# Autodesk Inventor assembly: (FINAL) 1QUAD WITH HARDWARE
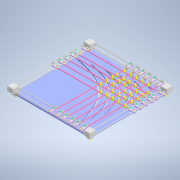
[picture p0: Inventor's stored thumbnail of the model, 180x180]
Saved by Autodesk Inventor 2022 (Build 260153000, 153)
## iProperties
Created: 2022-11-16
Part Number: (FINAL) 1QUAD WITH HARDWARE
Document SubType Name: Assembly
Designer: matia
Author: matia
## Documents named in this file (7)
- C:\Users\matia\Desktop\(V2) FULL ASSEMBLY\(FINAL) 1QUAD WITH HARDWARE.iam
- C:\Users\matia\Desktop\(V2) FULL ASSEMBLY\One quadrant Board.ipt
- C:\Users\matia\Desktop\(V2) FULL ASSEMBLY\bar.ipt
- C:\Users\matia\Desktop\(V2) FULL ASSEMBLY\(FINAL)2SIDEROLLER.iam
- C:\Users\matia\Desktop\(V2) FULL ASSEMBLY\newblockwithnopeg.ipt
- C:\Users\matia\Desktop\(V2) FULL ASSEMBLY\(FINAL) CORNER LH.iam
- C:\Users\matia\Desktop\(V2) FULL ASSEMBLY\(FINAL) CORNER RH.iam
## Components (55 placed, 6 different names)
1. One quadrant Board:1 — Mate:50, Mate:51, Mate:56, Mate:57, Mate:62, Mate:63, Mate:64, Mate:65
2. bar:1 — Mate:69, Mate:70
3. bar:2 — Mate:27, Mate:29, Mate:31, Mate:33, Mate:35, Mate:37, Mate:66, Mate:67
4. bar:3 — Mate:71, Mate:72
5. bar:4 — Mate:26, Mate:28, Mate:30, Mate:32, Mate:34, Mate:36, Mate:68, Mate:84, Mate:85
6. bar:5 — Mate:38, Mate:40, Mate:42, Mate:44, Mate:46, Mate:48, Mate:59, Mate:60
7. bar:6 — Mate:39, Mate:41, Mate:43, Mate:45, Mate:47, Mate:49, Mate:58, Mate:61
8. bar:7 — Mate:52, Mate:53
9. bar:8 — Mate:54, Mate:55
10. (FINAL)2SIDEROLLER:1 [sub-assembly] — Mate:26, Mate:27, Mate:80, Mate:100, Mate:110, Mate:114, Mate:134
11. (FINAL)2SIDEROLLER:2 [sub-assembly] — Mate:34, Mate:35, Mate:78, Mate:98, Mate:112, Mate:130, Mate:132
12. (FINAL)2SIDEROLLER:3 [sub-assembly] — Mate:36, Mate:37, Mate:82, Mate:102, Mate:104, Mate:106, Mate:108
13. (FINAL)2SIDEROLLER:4 [sub-assembly] — Mate:32, Mate:33, Mate:86, Mate:88, Mate:90, Mate:92, Mate:94
14. (FINAL)2SIDEROLLER:5 [sub-assembly] — Mate:30, Mate:31, Mate:74, Mate:116, Mate:118, Mate:120, Mate:122
15. (FINAL)2SIDEROLLER:6 [sub-assembly] — Mate:28, Mate:29, Mate:76, Mate:96, Mate:124, Mate:126, Mate:128
16. (FINAL)2SIDEROLLER:7 [sub-assembly] — Mate:38, Mate:39, Mate:87, Mate:103, Mate:109, Mate:111, Mate:115
17. (FINAL)2SIDEROLLER:8 [sub-assembly] — Mate:40, Mate:41, Mate:91, Mate:107, Mate:119, Mate:125, Mate:131
18. (FINAL)2SIDEROLLER:9 [sub-assembly] — Mate:42, Mate:43, Mate:93, Mate:121, Mate:127, Mate:129, Mate:133
19. (FINAL)2SIDEROLLER:10 [sub-assembly] — Mate:44, Mate:45, Mate:83, Mate:95, Mate:97, Mate:99, Mate:101
20. (FINAL)2SIDEROLLER:11 [sub-assembly] — Mate:46, Mate:47, Mate:89, Mate:105, Mate:113, Mate:117, Mate:123
21. (FINAL)2SIDEROLLER:12 [sub-assembly] — Mate:48, Mate:49, Mate:73, Mate:75, Mate:77, Mate:79, Mate:81
22. newblockwithnopeg:1 — Mate:73, Mate:74
23. (FINAL) CORNER LH:2 [sub-assembly] — Mate:56, Mate:57, Mate:58, Mate:59, Mate:60, Mate:61
24. (FINAL) CORNER LH:3 [sub-assembly] — Mate:64, Mate:65, Mate:69, Mate:70, Mate:71, Mate:72
25. (FINAL) CORNER RH:1 [sub-assembly] — Mate:50, Mate:51, Mate:52, Mate:53, Mate:54, Mate:55
26. (FINAL) CORNER RH:2 [sub-assembly] — Mate:62, Mate:63, Mate:66, Mate:67, Mate:68, Mate:84, Mate:85
27. newblockwithnopeg:2 — Mate:75, Mate:76
28. newblockwithnopeg:3 — Mate:81, Mate:82
29. newblockwithnopeg:4 — Mate:79, Mate:80
30. newblockwithnopeg:5 — Mate:77, Mate:78
31. newblockwithnopeg:6 — Mate:83, Mate:86
32. newblockwithnopeg:7 — Mate:87, Mate:88
33. newblockwithnopeg:8 — Mate:91, Mate:92
34. newblockwithnopeg:9 — Mate:89, Mate:90
35. newblockwithnopeg:10 — Mate:93, Mate:94
36. newblockwithnopeg:11 — Mate:95, Mate:96
37. newblockwithnopeg:12 — Mate:99, Mate:100
38. newblockwithnopeg:13 — Mate:97, Mate:98
39. newblockwithnopeg:14 — Mate:101, Mate:102
40. newblockwithnopeg:15 — Mate:103, Mate:104
41. newblockwithnopeg:16 — Mate:105, Mate:106
42. newblockwithnopeg:17 — Mate:115, Mate:116
43. newblockwithnopeg:18 — Mate:121, Mate:122
44. newblockwithnopeg:19 — Mate:125, Mate:126
45. newblockwithnopeg:20 — Mate:123, Mate:124
46. newblockwithnopeg:21 — Mate:119, Mate:120
47. newblockwithnopeg:22 — Mate:117, Mate:118
48. newblockwithnopeg:23 — Mate:113, Mate:114
49. newblockwithnopeg:24 — Mate:111, Mate:112
50. newblockwithnopeg:25 — Mate:109, Mate:110
51. newblockwithnopeg:26 — Mate:107, Mate:108
52. newblockwithnopeg:27 — Mate:133, Mate:134
53. newblockwithnopeg:28 — Mate:131, Mate:132
54. newblockwithnopeg:29 — Mate:129, Mate:130
55. newblockwithnopeg:30 — Mate:127, Mate:128
## Relationships (109: Mate 109)
- Mate:26: bar:4 ↔ (FINAL)2SIDEROLLER:1
- Mate:27: bar:2 ↔ (FINAL)2SIDEROLLER:1
- Mate:28: bar:4 ↔ (FINAL)2SIDEROLLER:6
- Mate:29: bar:2 ↔ (FINAL)2SIDEROLLER:6
- Mate:30: bar:4 ↔ (FINAL)2SIDEROLLER:5
- Mate:31: bar:2 ↔ (FINAL)2SIDEROLLER:5
- Mate:32: bar:4 ↔ (FINAL)2SIDEROLLER:4
- Mate:33: bar:2 ↔ (FINAL)2SIDEROLLER:4
- Mate:34: bar:4 ↔ (FINAL)2SIDEROLLER:2
- Mate:35: bar:2 ↔ (FINAL)2SIDEROLLER:2
- Mate:36: bar:4 ↔ (FINAL)2SIDEROLLER:3
- Mate:37: bar:2 ↔ (FINAL)2SIDEROLLER:3
- Mate:38: bar:5 ↔ (FINAL)2SIDEROLLER:7
- Mate:39: bar:6 ↔ (FINAL)2SIDEROLLER:7
- Mate:40: bar:5 ↔ (FINAL)2SIDEROLLER:8
- Mate:41: bar:6 ↔ (FINAL)2SIDEROLLER:8
- Mate:42: bar:5 ↔ (FINAL)2SIDEROLLER:9
- Mate:43: bar:6 ↔ (FINAL)2SIDEROLLER:9
- Mate:44: bar:5 ↔ (FINAL)2SIDEROLLER:10
- Mate:45: bar:6 ↔ (FINAL)2SIDEROLLER:10
- Mate:46: bar:5 ↔ (FINAL)2SIDEROLLER:11
- Mate:47: bar:6 ↔ (FINAL)2SIDEROLLER:11
- Mate:48: bar:5 ↔ (FINAL)2SIDEROLLER:12
- Mate:49: bar:6 ↔ (FINAL)2SIDEROLLER:12
- Mate:50: One quadrant Board:1 ↔ (FINAL) CORNER RH:1
- Mate:51: One quadrant Board:1 ↔ (FINAL) CORNER RH:1
- Mate:52: bar:7 ↔ (FINAL) CORNER RH:1
- Mate:53: bar:7 ↔ (FINAL) CORNER RH:1
- Mate:54: bar:8 ↔ (FINAL) CORNER RH:1
- Mate:55: bar:8 ↔ (FINAL) CORNER RH:1
- Mate:56: One quadrant Board:1 ↔ (FINAL) CORNER LH:2
- Mate:57: One quadrant Board:1 ↔ (FINAL) CORNER LH:2
- Mate:58: bar:6 ↔ (FINAL) CORNER LH:2
- Mate:59: bar:5 ↔ (FINAL) CORNER LH:2
- Mate:60: bar:5 ↔ (FINAL) CORNER LH:2
- Mate:61: bar:6 ↔ (FINAL) CORNER LH:2
- Mate:62: One quadrant Board:1 ↔ (FINAL) CORNER RH:2
- Mate:63: One quadrant Board:1 ↔ (FINAL) CORNER RH:2
- Mate:64: One quadrant Board:1 ↔ (FINAL) CORNER LH:3
- Mate:65: One quadrant Board:1 ↔ (FINAL) CORNER LH:3
- Mate:66: bar:2 ↔ (FINAL) CORNER RH:2
- Mate:67: bar:2 ↔ (FINAL) CORNER RH:2
- Mate:68: bar:4 ↔ (FINAL) CORNER RH:2
- Mate:69: bar:1 ↔ (FINAL) CORNER LH:3
- Mate:70: bar:1 ↔ (FINAL) CORNER LH:3
- Mate:71: bar:3 ↔ (FINAL) CORNER LH:3
- Mate:72: bar:3 ↔ (FINAL) CORNER LH:3
- Mate:73: (FINAL)2SIDEROLLER:12 ↔ newblockwithnopeg:1
- Mate:74: (FINAL)2SIDEROLLER:5 ↔ newblockwithnopeg:1
- Mate:75: (FINAL)2SIDEROLLER:12 ↔ newblockwithnopeg:2
- Mate:76: (FINAL)2SIDEROLLER:6 ↔ newblockwithnopeg:2
- Mate:77: (FINAL)2SIDEROLLER:12 ↔ newblockwithnopeg:5
- Mate:78: (FINAL)2SIDEROLLER:2 ↔ newblockwithnopeg:5
- Mate:79: (FINAL)2SIDEROLLER:12 ↔ newblockwithnopeg:4
- Mate:80: (FINAL)2SIDEROLLER:1 ↔ newblockwithnopeg:4
- Mate:81: (FINAL)2SIDEROLLER:12 ↔ newblockwithnopeg:3
- Mate:82: (FINAL)2SIDEROLLER:3 ↔ newblockwithnopeg:3
- Mate:83: (FINAL)2SIDEROLLER:10 ↔ newblockwithnopeg:6
- Mate:84: bar:4 ↔ (FINAL) CORNER RH:2
- Mate:85: bar:4 ↔ (FINAL) CORNER RH:2
- Mate:86: (FINAL)2SIDEROLLER:4 ↔ newblockwithnopeg:6
- Mate:87: (FINAL)2SIDEROLLER:7 ↔ newblockwithnopeg:7
- Mate:88: (FINAL)2SIDEROLLER:4 ↔ newblockwithnopeg:7
- Mate:89: (FINAL)2SIDEROLLER:11 ↔ newblockwithnopeg:9
- Mate:90: (FINAL)2SIDEROLLER:4 ↔ newblockwithnopeg:9
- Mate:91: (FINAL)2SIDEROLLER:8 ↔ newblockwithnopeg:8
- Mate:92: (FINAL)2SIDEROLLER:4 ↔ newblockwithnopeg:8
- Mate:93: (FINAL)2SIDEROLLER:9 ↔ newblockwithnopeg:10
- Mate:94: (FINAL)2SIDEROLLER:4 ↔ newblockwithnopeg:10
- Mate:95: (FINAL)2SIDEROLLER:10 ↔ newblockwithnopeg:11
- Mate:96: (FINAL)2SIDEROLLER:6 ↔ newblockwithnopeg:11
- Mate:97: (FINAL)2SIDEROLLER:10 ↔ newblockwithnopeg:13
- Mate:98: (FINAL)2SIDEROLLER:2 ↔ newblockwithnopeg:13
- Mate:99: (FINAL)2SIDEROLLER:10 ↔ newblockwithnopeg:12
- Mate:100: (FINAL)2SIDEROLLER:1 ↔ newblockwithnopeg:12
- Mate:101: (FINAL)2SIDEROLLER:10 ↔ newblockwithnopeg:14
- Mate:102: (FINAL)2SIDEROLLER:3 ↔ newblockwithnopeg:14
- Mate:103: (FINAL)2SIDEROLLER:7 ↔ newblockwithnopeg:15
- Mate:104: (FINAL)2SIDEROLLER:3 ↔ newblockwithnopeg:15
- Mate:105: (FINAL)2SIDEROLLER:11 ↔ newblockwithnopeg:16
- Mate:106: (FINAL)2SIDEROLLER:3 ↔ newblockwithnopeg:16
- Mate:107: (FINAL)2SIDEROLLER:8 ↔ newblockwithnopeg:26
- Mate:108: (FINAL)2SIDEROLLER:3 ↔ newblockwithnopeg:26
- Mate:109: (FINAL)2SIDEROLLER:7 ↔ newblockwithnopeg:25
- Mate:110: (FINAL)2SIDEROLLER:1 ↔ newblockwithnopeg:25
- Mate:111: (FINAL)2SIDEROLLER:7 ↔ newblockwithnopeg:24
- Mate:112: (FINAL)2SIDEROLLER:2 ↔ newblockwithnopeg:24
- Mate:113: (FINAL)2SIDEROLLER:11 ↔ newblockwithnopeg:23
- Mate:114: (FINAL)2SIDEROLLER:1 ↔ newblockwithnopeg:23
- Mate:115: (FINAL)2SIDEROLLER:7 ↔ newblockwithnopeg:17
- Mate:116: (FINAL)2SIDEROLLER:5 ↔ newblockwithnopeg:17
- Mate:117: (FINAL)2SIDEROLLER:11 ↔ newblockwithnopeg:22
- Mate:118: (FINAL)2SIDEROLLER:5 ↔ newblockwithnopeg:22
- Mate:119: (FINAL)2SIDEROLLER:8 ↔ newblockwithnopeg:21
- Mate:120: (FINAL)2SIDEROLLER:5 ↔ newblockwithnopeg:21
- Mate:121: (FINAL)2SIDEROLLER:9 ↔ newblockwithnopeg:18
- Mate:122: (FINAL)2SIDEROLLER:5 ↔ newblockwithnopeg:18
- Mate:123: (FINAL)2SIDEROLLER:11 ↔ newblockwithnopeg:20
- Mate:124: (FINAL)2SIDEROLLER:6 ↔ newblockwithnopeg:20
- Mate:125: (FINAL)2SIDEROLLER:8 ↔ newblockwithnopeg:19
- Mate:126: (FINAL)2SIDEROLLER:6 ↔ newblockwithnopeg:19
- Mate:127: (FINAL)2SIDEROLLER:9 ↔ newblockwithnopeg:30
- Mate:128: (FINAL)2SIDEROLLER:6 ↔ newblockwithnopeg:30
- Mate:129: (FINAL)2SIDEROLLER:9 ↔ newblockwithnopeg:29
- Mate:130: (FINAL)2SIDEROLLER:2 ↔ newblockwithnopeg:29
- Mate:131: (FINAL)2SIDEROLLER:8 ↔ newblockwithnopeg:28
- Mate:132: (FINAL)2SIDEROLLER:2 ↔ newblockwithnopeg:28
- Mate:133: (FINAL)2SIDEROLLER:9 ↔ newblockwithnopeg:27
- Mate:134: (FINAL)2SIDEROLLER:1 ↔ newblockwithnopeg:27
